# Autodesk Inventor assembly: Assembly Syringe
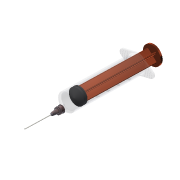
[picture p0: Inventor's stored thumbnail of the model, 180x180]
Saved by Autodesk Inventor 2018 (Build 220112000, 112)
## iProperties
Created: 2019-11-16
Part Number: Assembly Syringe
Document SubType Name: Assembly
Designer: ASUS
Author: ASUS
## Documents named in this file (5)
- C:\Users\ASUS\Pictures\Project Inventor\Assembly Syringe.iam
- C:\Users\ASUS\Pictures\Project Inventor\Plunger.ipt
- C:\Users\ASUS\Pictures\Project Inventor\Plunger Rubber.ipt
- C:\Users\ASUS\Pictures\Project Inventor\Body Syringe.ipt
- C:\Users\ASUS\Pictures\Project Inventor\Needle.ipt
## Components (4 placed, 4 different names)
1. Plunger:1 — Mate:1, Mate:2
2. Plunger Rubber:1 — Mate:1, Mate:2, Mate:3
3. Body Syringe:1 — Mate:3, Mate:4, Mate:5
4. Needle:1 — Mate:4, Mate:5
## Relationships (5: Mate 5)
- Mate:1: Plunger:1 ↔ Plunger Rubber:1
- Mate:2: Plunger:1 ↔ Plunger Rubber:1
- Mate:3: Plunger Rubber:1 ↔ Body Syringe:1
- Mate:4: Body Syringe:1 ↔ Needle:1
- Mate:5: Body Syringe:1 ↔ Needle:1
